# Autodesk Inventor assembly: shock_absorber
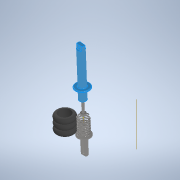
[picture p0: Inventor's stored thumbnail of the model, 180x180]
Saved by Autodesk Inventor 2022 (Build 260153000, 153)
## iProperties
Created: 2021-07-30
Part Number: shock_absorber
Document SubType Name: Assembly
Designer: Ian Kibandi
Author: Ian Kibandi
## Documents named in this file (7)
- C:\academics\YEAR 4\4.1\Manufacture Technology\Shock Absorber\shock_absorber.iam
- C:\academics\YEAR 4\4.1\Manufacture Technology\Shock Absorber\Air Suspension Air Bag.ipt
- C:\academics\YEAR 4\4.1\Manufacture Technology\Shock Absorber\Hydraulic fluid shield.ipt
- C:\academics\YEAR 4\4.1\Manufacture Technology\Shock Absorber\Piston Rod.ipt
- C:\academics\YEAR 4\4.1\Manufacture Technology\Shock Absorber\Piston.ipt
- C:\academics\YEAR 4\4.1\Manufacture Technology\Shock Absorber\shield.ipt
- C:\academics\YEAR 4\4.1\Manufacture Technology\Shock Absorber\spring.ipt
## Components (6 placed, 6 different names)
1. Air Suspension Air Bag:1
2. Hydraulic fluid shield:1 — Mate:2, Mate:5, Mate:6
3. Part2:1 — Insert:1, Rotation:1, Mate:3, Mate:4
4. Piston:1 — Insert:1
5. shield:1 — Rotation:1, Mate:2, Mate:3, Mate:4
6. spring:1 — Mate:5, Mate:6
## Relationships (7: Mate 5, Insert 1, RelateRotation 1)
- Insert:1: Part2:1 ↔ Piston:1
- Rotation:1 [RelateRotation] (1 ul): Part2:1 ↔ shield:1
- Mate:2: Hydraulic fluid shield:1 ↔ shield:1
- Mate:3: Part2:1 ↔ shield:1
- Mate:4: Part2:1 ↔ shield:1
- Mate:5: Hydraulic fluid shield:1 ↔ spring:1
- Mate:6: Hydraulic fluid shield:1 ↔ spring:1
